# Autodesk Inventor assembly: 42146-30
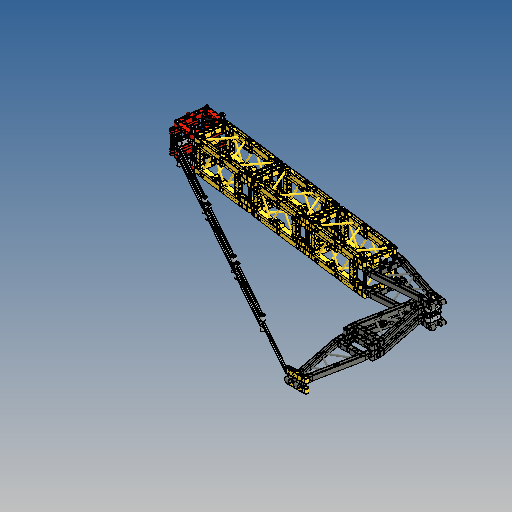
[picture p0: Inventor's stored thumbnail of the model, 512x512]
Saved by Autodesk Inventor 2025 (Build 290162010, 162A)
## iProperties
Created: 2024-12-05
Part Number: 42146-30
Material: Generisch
Document SubType Name: Assembly
Designer: hp.muther
Author: hp.muther
## Documents named in this file (33)
- D:\Inventor\Projekte\Muther\LEGO Technic\LEGO Technik - Raupenkran LR 13000 (42146)\42146-30.iam
- D:\Inventor\Projekte\Muther\LEGO Technic\LEGO Pieces\Rahmen, T-Stücke\79768-DkBluishGray.ipt
- D:\Inventor\Projekte\Muther\LEGO Technic\LEGO Pieces\Lochbalken\32316-Yellow.ipt
- D:\Inventor\Projekte\Muther\LEGO Technic\LEGO Pieces\Pin's\6558-Blue.ipt
- D:\Inventor\Projekte\Muther\LEGO Technic\LEGO Pieces\Verbindungselemente\2637-LtBluishGray.ipt
- D:\Inventor\Projekte\Muther\LEGO Technic\LEGO Pieces\Verbindungselemente\48989-LtBluishGray.ipt
- D:\Inventor\Projekte\Muther\LEGO Technic\LEGO Pieces\Achsen\4519-Yellow.ipt
- D:\Inventor\Projekte\Muther\LEGO Technic\LEGO Pieces\Diverses\61510-LtBluishGray.ipt
- D:\Inventor\Projekte\Muther\LEGO Technic\LEGO Pieces\Pin's\2780-Black.ipt
- D:\Inventor\Projekte\Muther\LEGO Technic\LEGO Pieces\Pin's\11214-Red.ipt
- D:\Inventor\Projekte\Muther\LEGO Technic\LEGO Pieces\Pin's\32054-LtBluishGray.ipt
- D:\Inventor\Projekte\Muther\LEGO Technic\LEGO Pieces\Lochbalken\32523-LtBluishGray.ipt
- D:\Inventor\Projekte\Muther\LEGO Technic\LEGO Pieces\Pin's\32556-Tan.ipt
- D:\Inventor\Projekte\Muther\LEGO Technic\LEGO Pieces\Verbindungselemente\39793-Yellow.ipt
- D:\Inventor\Projekte\Muther\LEGO Technic\LEGO Pieces\Rahmen, T-Stücke\79766-Yellow.ipt
- D:\Inventor\Projekte\Muther\LEGO Technic\LEGO Pieces\Rahmen, T-Stücke\79767-Yellow.ipt
- D:\Inventor\Projekte\Muther\LEGO Technic\LEGO Pieces\Pin's\43093-Blue.ipt
- D:\Inventor\Projekte\Muther\LEGO Technic\LEGO Pieces\Lochbalken\32524-LtBluishGray.ipt
- D:\Inventor\Projekte\Muther\LEGO Technic\LEGO Pieces\Achsen\44294-Yellow.ipt
- D:\Inventor\Projekte\Muther\LEGO Technic\LEGO Pieces\Achsen\32073-LtBluishGray.ipt
- D:\Inventor\Projekte\Muther\LEGO Technic\LEGO Pieces\Achsen\32062-Red.ipt
- D:\Inventor\Projekte\Muther\LEGO Technic\LEGO Pieces\Lochbalken schmal\11478-Black.ipt
- D:\Inventor\Projekte\Muther\LEGO Technic\LEGO Pieces\Lochbalken schmal\32063-Red.ipt
- D:\Inventor\Projekte\Muther\LEGO Technic\LEGO Pieces\Winkel\32526-LtBluishGray.ipt
- D:\Inventor\Projekte\Muther\LEGO Technic\LEGO Pieces\Rahmen, T-Stücke\64179-Red.ipt
- D:\Inventor\Projekte\Muther\LEGO Technic\LEGO Pieces\Pin's\4274-Red.ipt
- D:\Inventor\Projekte\Muther\LEGO Technic\LEGO Pieces\Steine rund\58176-TransRed.ipt
- D:\Inventor\Projekte\Muther\LEGO Technic\LEGO Pieces\Räder, Raupe\42610-LtBluishGray.ipt
- D:\Inventor\Projekte\Muther\LEGO Technic\LEGO Pieces\Rund\3713-LtBluishGray.ipt
- D:\Inventor\Projekte\Muther\LEGO Technic\LEGO Pieces\Rund\6538c-Red.ipt
- D:\Inventor\Projekte\Muther\LEGO Technic\LEGO Pieces\Achsen\99008-Tan.ipt
- D:\Inventor\Projekte\Muther\LEGO Technic\LEGO Pieces\Verbindungselemente\6575-Black.ipt
- D:\Inventor\Projekte\Muther\LEGO Technic\LEGO Pieces\Achsen\87083-DkBluishGray.ipt
## Components (163 placed, 32 different names)
1. 79768-DkBluishGray:1 — Einfügen:6, Passend:1, Einfügen:18, Einfügen:24, Passend:7, Einfügen:27
2. 32316-Yellow:1 — Einfügen:1, Einfügen:2, Einfügen:3, Einfügen:5, Einfügen:6, Passend:5
3. 6558-Blue:1 — Einfügen:1
4. 6558-Blue:2 — Einfügen:2
5. 6558-Blue:3 — Einfügen:3, Passend:1
6. 6558-Blue:4 — Einfügen:4
7. 2637-LtBluishGray:1 — Einfügen:4, Einfügen:5, Einfügen:180, Fluchtend:51
8. 32316-Yellow:2 — Einfügen:18, Passend:5
9. 79768-DkBluishGray:2 — Einfügen:21, Einfügen:22, Einfügen:23, Passend:6, Einfügen:24, Einfügen:26
10. 79768-DkBluishGray:3 — Einfügen:27, Passend:8, Einfügen:28
11. 48989-LtBluishGray:1 — Einfügen:23, Passend:6
12. 6558-Blue:5 — Einfügen:21, Passend:7, Passend:8
13. 6558-Blue:6 — Einfügen:22
14. 4519-Yellow:1 — Einfügen:25
15. 61510-LtBluishGray:1 — Einfügen:25, Einfügen:26
16. 2780-Black:1 — Einfügen:28
17. 79768-DkBluishGray:4 — Passend:17
18. 11214-Red:1
19. 32054-LtBluishGray:1
20. 32523-LtBluishGray:1
21. 2780-Black:2
22. 11214-Red:2
23. 32054-LtBluishGray:2
24. 32523-LtBluishGray:2
25. 2780-Black:3
26. 2780-Black:4
27. 2780-Black:5
28. 2780-Black:6
29. 32556-Tan:1
30. 39793-Yellow:1
31. 79768-DkBluishGray:5 — Einfügen:70
32. 32556-Tan:2
33. 79766-Yellow:1 — Einfügen:112
34. 79767-Yellow:1
35. 2780-Black:7 — Passend:25
36. 2780-Black:8
37. 2780-Black:9
38. 2780-Black:10
39. 2780-Black:11
40. 2780-Black:12
41. 2780-Black:13
42. 43093-Blue:1
43. 43093-Blue:2
44. 79766-Yellow:2 — Einfügen:71, Einfügen:72
45. 79767-Yellow:2
46. 2780-Black:14
47. 2780-Black:15
48. 2780-Black:16
49. 2780-Black:17
50. 2780-Black:18
51. 2780-Black:19
52. 2780-Black:20
53. 43093-Blue:3
54. 43093-Blue:4
55. 2780-Black:21
56. 2780-Black:22
57. 2780-Black:23 — Passend:17
58. 32524-LtBluishGray:1 — Einfügen:70
59. 44294-Yellow:1 — Einfügen:72
60. 44294-Yellow:2 — Einfügen:71
61. 79766-Yellow:3
62. 79767-Yellow:3
63. 2780-Black:24
64. 2780-Black:25
65. 2780-Black:26
66. 2780-Black:27
67. 2780-Black:28
68. 2780-Black:29
69. 43093-Blue:5
70. 43093-Blue:6
71. 79766-Yellow:4 — Einfügen:114, Einfügen:115, Einfügen:171
72. 79767-Yellow:4 — Tangential:1
73. 2780-Black:30
74. 2780-Black:31 — Passend:43
75. 2780-Black:32
76. 2780-Black:33
77. 2780-Black:34
78. 2780-Black:35
79. 43093-Blue:7
80. 43093-Blue:8
81. 79766-Yellow:5 — Einfügen:112, Passend:25
82. 2780-Black:36
83. 2780-Black:37
84. 2780-Black:38
85. 2780-Black:39
86. 2780-Black:40
87. 2780-Black:41
88. 43093-Blue:9
89. 43093-Blue:10
90. 79767-Yellow:5
91. 79766-Yellow:6 — Einfügen:113, Einfügen:116
92. 2780-Black:42
93. 2780-Black:43
94. 2780-Black:44
95. 2780-Black:45
96. 2780-Black:46
97. 2780-Black:47
98. 43093-Blue:11
99. 43093-Blue:12
100. 79767-Yellow:6
101. 44294-Yellow:3 — Einfügen:113
102. 44294-Yellow:4 — Einfügen:114
103. 44294-Yellow:5 — Einfügen:115
104. 44294-Yellow:6 — Einfügen:116
105. 32073-LtBluishGray:1 — Einfügen:156, Passend:40
106. 32062-Red:1 — Einfügen:122
107. 4519-Yellow:2 — Einfügen:144, Einfügen:145
108. 44294-Yellow:7 — Einfügen:147
109. 32073-LtBluishGray:2 — Einfügen:123, Passend:31, Passend:32
110. 32316-Yellow:3 — Einfügen:118, Einfügen:120, Einfügen:121, Passend:31
111. 11478-Black:1 — Einfügen:117, Passend:26, Einfügen:121
112. 32063-Red:1 — Einfügen:117, Passend:26, Passend:32, Einfügen:133, Einfügen:134, Einfügen:136, Einfügen:159
113. 6558-Blue:7 — Einfügen:118
114. 11478-Black:2 — Einfügen:120, Einfügen:122, Einfügen:123
115. 32063-Red:2 — Einfügen:131, Einfügen:132, Einfügen:135, Einfügen:137
116. 6558-Blue:8 — Einfügen:131, Passend:34, Passend:36
117. 6558-Blue:9 — Einfügen:132
118. 6558-Blue:10 — Einfügen:133, Passend:33
119. 6558-Blue:11 — Einfügen:134, Passend:42
120. 32523-LtBluishGray:3 — Einfügen:136, Passend:33, Einfügen:161
121. 32526-LtBluishGray:1 — Einfügen:137, Einfügen:141, Einfügen:156, Einfügen:157, Fluchtend:1, Tangential:1
122. 32523-LtBluishGray:4 — Einfügen:135, Passend:34
123. 64179-Red:1 — Einfügen:141, Passend:36, Einfügen:143, Passend:37, Einfügen:170, Einfügen:171, Passend:43, Einfügen:174, Einfügen:175, Winkel:3
124. 4274-Red:1
125. 58176-TransRed:1
126. 32063-Red:3 — Einfügen:140, Passend:35, Einfügen:146, Einfügen:150, Einfügen:181
127. 32063-Red:4 — Einfügen:140, Passend:35, Einfügen:142, Einfügen:143, Passend:37
128. 2780-Black:48 — Einfügen:142
129. 32054-LtBluishGray:3 — Einfügen:144, Einfügen:146
130. 32054-LtBluishGray:4 — Einfügen:145
131. 42610-LtBluishGray:1 — Einfügen:148
132. 42610-LtBluishGray:2 — Einfügen:149, Einfügen:150
133. 3713-LtBluishGray:1 — Einfügen:147, Einfügen:148, Einfügen:149
134. 64179-Red:2 — Einfügen:155, Passend:39, Einfügen:161, Passend:42, Einfügen:172, Einfügen:173
135. 4274-Red:2
136. 58176-TransRed:2
137. 32063-Red:5
138. 32063-Red:6 — Einfügen:155, Passend:39
139. 2780-Black:49
140. 2637-LtBluishGray:2 — Einfügen:157, Einfügen:158, Passend:41, Fluchtend:52, Passend:52, Passend:53
141. 3713-LtBluishGray:2 — Einfügen:158, Passend:40, Einfügen:160
142. 32526-LtBluishGray:2 — Einfügen:159, Fluchtend:1
143. 2637-LtBluishGray:3 — Einfügen:160, Passend:41
144. 6538c-Red:1 — Einfügen:162, Einfügen:163, Einfügen:164, Einfügen:165
145. 99008-Tan:1 — Einfügen:162
146. 99008-Tan:2 — Einfügen:163
147. 32073-LtBluishGray:3 — Einfügen:168, Winkel:3
148. 32073-LtBluishGray:4 — Einfügen:169
149. 42610-LtBluishGray:3 — Einfügen:164, Einfügen:166
150. 42610-LtBluishGray:4 — Einfügen:165, Einfügen:167
151. 6575-Black:1 — Einfügen:166
152. 6575-Black:2 — Einfügen:167, Einfügen:168, Einfügen:169, Einfügen:170
153. 32054-LtBluishGray:5 — Einfügen:172
154. 32054-LtBluishGray:6 — Einfügen:175
155. 32054-LtBluishGray:7 — Einfügen:173
156. 32054-LtBluishGray:8 — Einfügen:174
157. 2637-LtBluishGray:4 — Passend:51
158. 2637-LtBluishGray:5 — Einfügen:177, Passend:51, Einfügen:180, Fluchtend:51
159. 48989-LtBluishGray:2 — Einfügen:177, Einfügen:178, Fluchtend:50
160. 2637-LtBluishGray:6 — Passend:50
161. 2637-LtBluishGray:7 — Einfügen:178, Einfügen:179, Fluchtend:52
162. 48989-LtBluishGray:3 — Einfügen:179, Fluchtend:50, Passend:50, Passend:52, Passend:53
163. 87083-DkBluishGray:1 — Einfügen:181
## Relationships (214: Insert 161, Mate 46, Flush 4, Angle 2, Tangent 1)
- Einfügen:112 [Insert]: 79766-Yellow:1 ↔ 79766-Yellow:5
- Passend:52 [Mate]: 2637-LtBluishGray:2 ↔ 48989-LtBluishGray:3
- Passend:53 [Mate] (-240 mm): 2637-LtBluishGray:2 ↔ 48989-LtBluishGray:3
- Einfügen:1 [Insert]: 32316-Yellow:1 ↔ 6558-Blue:1
- Einfügen:2 [Insert]: 32316-Yellow:1 ↔ 6558-Blue:2
- Einfügen:3 [Insert]: 32316-Yellow:1 ↔ 6558-Blue:3
- Einfügen:4 [Insert]: 6558-Blue:4 ↔ 2637-LtBluishGray:1
- Einfügen:5 [Insert]: 32316-Yellow:1 ↔ 2637-LtBluishGray:1
- Einfügen:6 [Insert]: 79768-DkBluishGray:1 ↔ 32316-Yellow:1
- Passend:1 [Mate]: 79768-DkBluishGray:1 ↔ 6558-Blue:3
- Einfügen:18 [Insert]: 79768-DkBluishGray:1 ↔ 32316-Yellow:2
- Passend:5 [Mate]: 32316-Yellow:1 ↔ 32316-Yellow:2
- Einfügen:21 [Insert]: 79768-DkBluishGray:2 ↔ 6558-Blue:5
- Einfügen:22 [Insert]: 79768-DkBluishGray:2 ↔ 6558-Blue:6
- Einfügen:23 [Insert]: 79768-DkBluishGray:2 ↔ 48989-LtBluishGray:1
- Passend:6 [Mate]: 79768-DkBluishGray:2 ↔ 48989-LtBluishGray:1
- Einfügen:24 [Insert]: 79768-DkBluishGray:1 ↔ 79768-DkBluishGray:2
- Passend:7 [Mate]: 79768-DkBluishGray:1 ↔ 6558-Blue:5
- Einfügen:25 [Insert] (-16 mm): 4519-Yellow:1 ↔ 61510-LtBluishGray:1
- Einfügen:26 [Insert]: 79768-DkBluishGray:2 ↔ 61510-LtBluishGray:1
- Einfügen:27 [Insert]: 79768-DkBluishGray:1 ↔ 79768-DkBluishGray:3
- Passend:8 [Mate]: 79768-DkBluishGray:3 ↔ 6558-Blue:5
- Einfügen:28 [Insert]: 79768-DkBluishGray:3 ↔ 2780-Black:1
- [Insert]: 79768-DkBluishGray:2 ↔ 79768-DkBluishGray:4
- [Insert]: 79768-DkBluishGray:4 ↔ 2780-Black:2
- [Insert]: 11214-Red:1 ↔ 32054-LtBluishGray:1
- [Insert]: 32054-LtBluishGray:1 ↔ 32523-LtBluishGray:1
- [Insert]: 11214-Red:2 ↔ 32054-LtBluishGray:2
- [Insert]: 32523-LtBluishGray:1 ↔ 32054-LtBluishGray:2
- [Insert]: 32054-LtBluishGray:1 ↔ 32523-LtBluishGray:2
- [Mate]: 11214-Red:2 ↔ 32523-LtBluishGray:2
- [Insert]: 79768-DkBluishGray:4 ↔ 32523-LtBluishGray:1
- [Mate]: 79768-DkBluishGray:4 ↔ 32054-LtBluishGray:2
- [Insert]: 2780-Black:6 ↔ 39793-Yellow:1
- [Insert]: 2780-Black:5 ↔ 39793-Yellow:1
- [Insert]: 2780-Black:4 ↔ 39793-Yellow:1
- [Insert]: 2780-Black:3 ↔ 39793-Yellow:1
- [Insert]: 79768-DkBluishGray:4 ↔ 32556-Tan:1
- [Insert]: 79768-DkBluishGray:4 ↔ 39793-Yellow:1
- [Mate]: 79768-DkBluishGray:4 ↔ 2780-Black:4
- [Insert]: 79768-DkBluishGray:5 ↔ 32556-Tan:2
- [Insert]: 39793-Yellow:1 ↔ 79768-DkBluishGray:5
- [Mate]: 2780-Black:5 ↔ 79768-DkBluishGray:5
- [Insert]: 79766-Yellow:1 ↔ 43093-Blue:2
- [Insert]: 79766-Yellow:1 ↔ 43093-Blue:1
- [Insert]: 79766-Yellow:1 ↔ 2780-Black:8
- [Insert]: 79766-Yellow:1 ↔ 2780-Black:7
- [Insert]: 79766-Yellow:1 ↔ 2780-Black:9
- [Insert]: 79766-Yellow:1 ↔ 2780-Black:11
- [Insert]: 79766-Yellow:1 ↔ 2780-Black:13
- [Insert]: 79766-Yellow:1 ↔ 2780-Black:12
- [Insert]: 79766-Yellow:1 ↔ 2780-Black:10
- [Insert]: 79766-Yellow:1 ↔ 79767-Yellow:1
- [Mate]: 79767-Yellow:1 ↔ 2780-Black:12
- [Insert]: 79766-Yellow:2 ↔ 43093-Blue:4
- [Insert]: 79766-Yellow:2 ↔ 43093-Blue:3
- [Insert]: 79766-Yellow:2 ↔ 2780-Black:15
- [Insert]: 79766-Yellow:2 ↔ 2780-Black:14
- [Insert]: 79766-Yellow:2 ↔ 2780-Black:16
- [Insert]: 79766-Yellow:2 ↔ 2780-Black:18
- [Insert]: 79766-Yellow:2 ↔ 2780-Black:20
- [Insert]: 79766-Yellow:2 ↔ 2780-Black:19
- [Insert]: 79766-Yellow:2 ↔ 2780-Black:17
- [Insert]: 79766-Yellow:2 ↔ 79767-Yellow:2
- [Mate]: 79767-Yellow:2 ↔ 2780-Black:19
- [Insert]: 79766-Yellow:1 ↔ 79767-Yellow:2
- [Mate]: 2780-Black:13 ↔ 79767-Yellow:2
- [Insert]: 2780-Black:21 ↔ 32524-LtBluishGray:1
- [Insert]: 2780-Black:22 ↔ 32524-LtBluishGray:1
- [Insert]: 2780-Black:23 ↔ 32524-LtBluishGray:1
- [Insert]: 79766-Yellow:2 ↔ 32524-LtBluishGray:1
- [Mate]: 2780-Black:9 ↔ 32524-LtBluishGray:1
- Einfügen:70 [Insert]: 79768-DkBluishGray:5 ↔ 32524-LtBluishGray:1
- Passend:17 [Mate]: 79768-DkBluishGray:4 ↔ 2780-Black:23
- Einfügen:71 [Insert]: 79766-Yellow:2 ↔ 44294-Yellow:2
- Einfügen:72 [Insert]: 79766-Yellow:2 ↔ 44294-Yellow:1
- [Insert]: 79766-Yellow:3 ↔ 43093-Blue:6
- [Insert]: 79766-Yellow:3 ↔ 43093-Blue:5
- [Insert]: 79766-Yellow:3 ↔ 2780-Black:25
- [Insert]: 79766-Yellow:3 ↔ 2780-Black:24
- [Insert]: 79766-Yellow:3 ↔ 2780-Black:27
- [Insert]: 79766-Yellow:3 ↔ 2780-Black:29
- [Insert]: 79766-Yellow:3 ↔ 2780-Black:28
- [Insert]: 79766-Yellow:3 ↔ 2780-Black:26
- [Insert]: 79766-Yellow:3 ↔ 79767-Yellow:3
- [Mate]: 79767-Yellow:3 ↔ 2780-Black:28
- [Insert]: 79766-Yellow:4 ↔ 43093-Blue:8
- [Insert]: 79766-Yellow:4 ↔ 43093-Blue:7
- [Insert]: 79766-Yellow:4 ↔ 2780-Black:31
- [Insert]: 79766-Yellow:4 ↔ 2780-Black:30
- [Insert]: 79766-Yellow:4 ↔ 2780-Black:33
- [Insert]: 79766-Yellow:4 ↔ 2780-Black:35
- [Insert]: 79766-Yellow:4 ↔ 2780-Black:34
- [Insert]: 79766-Yellow:4 ↔ 2780-Black:32
- [Insert]: 79766-Yellow:4 ↔ 79767-Yellow:4
- [Mate]: 79767-Yellow:4 ↔ 2780-Black:34
- [Insert]: 79766-Yellow:3 ↔ 79767-Yellow:4
- [Mate]: 2780-Black:29 ↔ 79767-Yellow:4
- [Insert]: 79766-Yellow:5 ↔ 43093-Blue:10
- [Insert]: 79766-Yellow:5 ↔ 43093-Blue:9
- [Insert]: 79766-Yellow:5 ↔ 2780-Black:37
- [Insert]: 79766-Yellow:5 ↔ 2780-Black:36
- [Insert]: 79766-Yellow:5 ↔ 2780-Black:39
- [Insert]: 79766-Yellow:5 ↔ 2780-Black:41
- [Insert]: 79766-Yellow:5 ↔ 2780-Black:40
- [Insert]: 79766-Yellow:5 ↔ 2780-Black:38
- [Insert]: 79766-Yellow:5 ↔ 79767-Yellow:5
- [Insert]: 79766-Yellow:6 ↔ 43093-Blue:12
- [Insert]: 79766-Yellow:6 ↔ 43093-Blue:11
- [Insert]: 79766-Yellow:6 ↔ 2780-Black:43
- [Insert]: 79766-Yellow:6 ↔ 2780-Black:42
- [Insert]: 79766-Yellow:6 ↔ 2780-Black:45
- [Insert]: 79766-Yellow:6 ↔ 2780-Black:47
- [Insert]: 79766-Yellow:6 ↔ 2780-Black:46
- [Insert]: 79766-Yellow:6 ↔ 2780-Black:44
- [Insert]: 79766-Yellow:6 ↔ 79767-Yellow:6
- [Insert]: 79766-Yellow:5 ↔ 79767-Yellow:6
- [Mate]: 2780-Black:41 ↔ 79767-Yellow:5
- [Mate]: 2780-Black:40 ↔ 79767-Yellow:6
- [Mate]: 2780-Black:47 ↔ 79767-Yellow:6
- [Insert]: 79766-Yellow:4 ↔ 79766-Yellow:6
- [Mate]: 79766-Yellow:4 ↔ 2780-Black:42
- Passend:25 [Mate]: 2780-Black:7 ↔ 79766-Yellow:5
- Einfügen:113 [Insert]: 79766-Yellow:6 ↔ 44294-Yellow:3
- Einfügen:114 [Insert]: 79766-Yellow:4 ↔ 44294-Yellow:4
- Einfügen:115 [Insert]: 79766-Yellow:4 ↔ 44294-Yellow:5
- Einfügen:116 [Insert]: 79766-Yellow:6 ↔ 44294-Yellow:6
- Einfügen:117 [Insert]: 11478-Black:1 ↔ 32063-Red:1
- Passend:26 [Mate]: 11478-Black:1 ↔ 32063-Red:1
- Einfügen:118 [Insert]: 32316-Yellow:3 ↔ 6558-Blue:7
- [Insert]: 11478-Black:2 ↔ 32063-Red:2
- [Mate]: 11478-Black:2 ↔ 32063-Red:2
- Einfügen:120 [Insert]: 32316-Yellow:3 ↔ 11478-Black:2
- Einfügen:121 [Insert]: 32316-Yellow:3 ↔ 11478-Black:1
- Einfügen:122 [Insert]: 32062-Red:1 ↔ 11478-Black:2
- Einfügen:123 [Insert] (-28 mm): 32073-LtBluishGray:2 ↔ 11478-Black:2
- Passend:31 [Mate]: 32073-LtBluishGray:2 ↔ 32316-Yellow:3
- Passend:32 [Mate]: 32073-LtBluishGray:2 ↔ 32063-Red:1
- Einfügen:131 [Insert]: 32063-Red:2 ↔ 6558-Blue:8
- Einfügen:132 [Insert]: 32063-Red:2 ↔ 6558-Blue:9
- Einfügen:133 [Insert]: 32063-Red:1 ↔ 6558-Blue:10
- Einfügen:134 [Insert]: 32063-Red:1 ↔ 6558-Blue:11
- Einfügen:135 [Insert]: 32063-Red:2 ↔ 32523-LtBluishGray:4
- Einfügen:136 [Insert]: 32063-Red:1 ↔ 32523-LtBluishGray:3
- Passend:33 [Mate]: 6558-Blue:10 ↔ 32523-LtBluishGray:3
- Passend:34 [Mate]: 6558-Blue:8 ↔ 32523-LtBluishGray:4
- Einfügen:137 [Insert]: 32063-Red:2 ↔ 32526-LtBluishGray:1
- [Insert]: 4274-Red:1 ↔ 58176-TransRed:1
- [Insert]: 64179-Red:1 ↔ 4274-Red:1
- Einfügen:140 [Insert]: 32063-Red:3 ↔ 32063-Red:4
- Passend:35 [Mate]: 32063-Red:3 ↔ 32063-Red:4
- Einfügen:141 [Insert]: 32526-LtBluishGray:1 ↔ 64179-Red:1
- Passend:36 [Mate]: 6558-Blue:8 ↔ 64179-Red:1
- Einfügen:142 [Insert]: 32063-Red:4 ↔ 2780-Black:48
- Einfügen:143 [Insert]: 64179-Red:1 ↔ 32063-Red:4
- Passend:37 [Mate]: 64179-Red:1 ↔ 32063-Red:4
- Einfügen:144 [Insert] (-8 mm): 4519-Yellow:2 ↔ 32054-LtBluishGray:3
- Einfügen:145 [Insert] (-8 mm): 4519-Yellow:2 ↔ 32054-LtBluishGray:4
- Einfügen:146 [Insert]: 32063-Red:3 ↔ 32054-LtBluishGray:3
- Einfügen:147 [Insert] (-32 mm): 44294-Yellow:7 ↔ 3713-LtBluishGray:1
- Einfügen:148 [Insert]: 42610-LtBluishGray:1 ↔ 3713-LtBluishGray:1
- Einfügen:149 [Insert]: 42610-LtBluishGray:2 ↔ 3713-LtBluishGray:1
- Einfügen:150 [Insert]: 32063-Red:3 ↔ 42610-LtBluishGray:2
- [Insert]: 4274-Red:2 ↔ 58176-TransRed:2
- [Insert]: 64179-Red:2 ↔ 4274-Red:2
- [Insert]: 32063-Red:5 ↔ 32063-Red:6
- [Mate]: 32063-Red:5 ↔ 32063-Red:6
- [Insert]: 32063-Red:6 ↔ 2780-Black:49
- Einfügen:155 [Insert]: 64179-Red:2 ↔ 32063-Red:6
- Passend:39 [Mate]: 64179-Red:2 ↔ 32063-Red:6
- Einfügen:156 [Insert]: 32073-LtBluishGray:1 ↔ 32526-LtBluishGray:1
- Einfügen:157 [Insert]: 32526-LtBluishGray:1 ↔ 2637-LtBluishGray:2
- Einfügen:158 [Insert]: 2637-LtBluishGray:2 ↔ 3713-LtBluishGray:2
- Passend:40 [Mate]: 32073-LtBluishGray:1 ↔ 3713-LtBluishGray:2
- Einfügen:159 [Insert]: 32063-Red:1 ↔ 32526-LtBluishGray:2
- Einfügen:160 [Insert]: 3713-LtBluishGray:2 ↔ 2637-LtBluishGray:3
- Fluchtend:1 [Flush]: 32526-LtBluishGray:1 ↔ 32526-LtBluishGray:2
- Passend:41 [Mate]: 2637-LtBluishGray:2 ↔ 2637-LtBluishGray:3
- Einfügen:161 [Insert]: 32523-LtBluishGray:3 ↔ 64179-Red:2
- Passend:42 [Mate]: 6558-Blue:11 ↔ 64179-Red:2
- Einfügen:162 [Insert]: 6538c-Red:1 ↔ 99008-Tan:1
- Einfügen:163 [Insert]: 6538c-Red:1 ↔ 99008-Tan:2
- Einfügen:164 [Insert]: 6538c-Red:1 ↔ 42610-LtBluishGray:3
- Einfügen:165 [Insert]: 6538c-Red:1 ↔ 42610-LtBluishGray:4
- Einfügen:166 [Insert]: 42610-LtBluishGray:3 ↔ 6575-Black:1
- Einfügen:167 [Insert]: 42610-LtBluishGray:4 ↔ 6575-Black:2
- Einfügen:168 [Insert]: 32073-LtBluishGray:3 ↔ 6575-Black:2
- Einfügen:169 [Insert]: 32073-LtBluishGray:4 ↔ 6575-Black:2
- Einfügen:170 [Insert]: 64179-Red:1 ↔ 6575-Black:2
- Einfügen:171 [Insert]: 79766-Yellow:4 ↔ 64179-Red:1
- Passend:43 [Mate]: 2780-Black:31 ↔ 64179-Red:1
- Einfügen:172 [Insert]: 64179-Red:2 ↔ 32054-LtBluishGray:5
- Einfügen:173 [Insert]: 64179-Red:2 ↔ 32054-LtBluishGray:7
- Einfügen:174 [Insert]: 64179-Red:1 ↔ 32054-LtBluishGray:8
- Einfügen:175 [Insert]: 64179-Red:1 ↔ 32054-LtBluishGray:6
- [Mate] (8 mm): 2637-LtBluishGray:4 ↔ 48989-LtBluishGray:2
- [Mate]: 2637-LtBluishGray:4 ↔ 2637-LtBluishGray:5
- [Angle] (0 deg): 2637-LtBluishGray:4 ↔ 48989-LtBluishGray:2
- [Insert]: 48989-LtBluishGray:2 ↔ 2637-LtBluishGray:6
- [Mate]: 48989-LtBluishGray:2 ↔ 2637-LtBluishGray:7
- [Mate]: 2637-LtBluishGray:4 ↔ 48989-LtBluishGray:2
- [Mate]: 2637-LtBluishGray:4 ↔ 48989-LtBluishGray:2
- Einfügen:177 [Insert]: 2637-LtBluishGray:5 ↔ 48989-LtBluishGray:2
- Einfügen:178 [Insert]: 48989-LtBluishGray:2 ↔ 2637-LtBluishGray:7
- Einfügen:179 [Insert]: 2637-LtBluishGray:7 ↔ 48989-LtBluishGray:3
- Fluchtend:50 [Flush]: 48989-LtBluishGray:2 ↔ 48989-LtBluishGray:3
- Passend:50 [Mate]: 2637-LtBluishGray:6 ↔ 48989-LtBluishGray:3
- Passend:51 [Mate]: 2637-LtBluishGray:4 ↔ 2637-LtBluishGray:5
- Einfügen:180 [Insert]: 2637-LtBluishGray:1 ↔ 2637-LtBluishGray:5
- Fluchtend:51 [Flush]: 2637-LtBluishGray:1 ↔ 2637-LtBluishGray:5
- Fluchtend:52 [Flush]: 2637-LtBluishGray:2 ↔ 2637-LtBluishGray:7
- Tangential:1: 79767-Yellow:4 ↔ 32526-LtBluishGray:1
- Einfügen:181 [Insert]: 32063-Red:3 ↔ 87083-DkBluishGray:1
- Winkel:3 [Angle] (0 deg): 64179-Red:1 ↔ 32073-LtBluishGray:3
## Named parameters: d797_d10 = 0 deg, d809_d0 = 0 mm, d38_d4 = 0 mm, d39_d5 = 0 mm, d40_d6 = 0 mm, d16_d13 = 0 mm, d53_d0 = 0 mm, d54_d1 = 0 mm, d55_d2 = 0 mm, d3_d1 = 0 mm, d57_d4 = 0 mm, d58_d5 = 0 mm, d59_d6 = 0 mm, d60_d7 = 0 mm, d61_d8 = 0 mm, d62_d9 = 0 mm, d63_d10 = 0 mm, d11_d0 = 0 mm, d12_d9 = 0 mm, d13_d10 = 0 mm, d14_d1 = 0 mm, d15_d2 = 0 mm, d16_d3 = 0 mm, d17_d4 = 0 mm, d18_d5 = 0 mm, d19_d6 = 0 mm, d20_d7 = 0 mm, d21_d8 = 0 mm, d75_d22 = 0 mm, d78_d25 = 0 mm, d79_d26 = 0 mm, d80_d27 = 0 mm, d81_d28 = 0 mm, d82_d0 = 0 mm, d83_d1 = 0 mm, d84_d2 = 0 mm, d85_d3 = 0 mm, d90_d5 = 0 mm, d91_d6 = 0 mm, d92_d7 = 0 mm, d93_d8 = 0 mm, d94_d9 = 0 mm, d95_d10 = 0 mm, d96_d11_d0 = 0 mm, d97_d12_d9 = 0 mm, d98_d13_d10 = 0 mm, d99_d14_d1 = 0 mm, d100_d15_d2 = 0 mm, d101_d16_d3 = 0 mm, d102_d18_d5 = 0 mm, d103_d19_d6 = 0 mm, d104_d20_d7 = 0 mm, d105_d21_d8 = 0 mm, d106_d22 = 0 mm, d107_d23 = 0 mm, d39_d38 = 0 mm, d40_d30_d5 = 0 mm, d41_d31_d6 = 0 mm, d42_d32_d7 = 0 mm, d43_d33_d8 = 0 mm, d44_d34_d0 = 0 mm, d45_d35_d1 = 0 mm, d46_d36_d2 = 0 mm, d47_d37_d3 = 0 mm, d30_d5 = 0 mm, d31_d6 = 0 mm, d32_d7 = 0 mm, d33_d8 = 0 mm, d34_d0 = 0 mm, d35_d1 = 0 mm, d36_d2 = 0 mm, d37_d3 = 0 mm, d132_d0 = 0 mm, d133_d1 = 0 mm, d134_d2 = 0 mm, d135_d3 = 0 mm, d145_d142 = 0 mm, d146_d143 = 0 mm, d6_d3 = 0 mm, d794_d7 = 0 mm, d188_d178 = 0 mm, d189_d179 = 0 mm, d190_d180 = 0 mm, d192_d6_d3 = 0 mm, d193_d794_d7 = 0 mm, d194_d174 = 0 mm, d195_d175 = 0 mm
